# Autodesk Inventor assembly: SHPSNA5
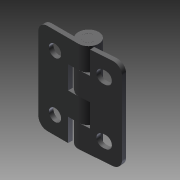
[picture p0: Inventor's stored thumbnail of the model, 180x180]
Saved by Autodesk Inventor 2015 SP1 (Build 190203100, 203)
## iProperties
Category: PARTsolutions
Company: MISUMI
Created: 2015-01-26
Part Number: SHPSNA5
Catalog Web Link: www.cadenas.de
Description: SHPSNA-Hinges with Slotted Holes
Vendor: MISUMI
Document SubType Name: Assembly
Designer: PARTuser1
Manufacturer: MISUMI
PSOL_IDENT_0: {\\10.0.0.236\data_v8\23d-libs\misumi\metric\44_handles_hinges\shpsna_asmtab.prj},161 {VTYP=3D},{STY
PSOL_IDENT_1: P=ASSTAB},{NB=SHPSNA5},{LINA=SHPSNA5},{NN=SHPSNA},{DATE=14.11.2014 09:15:25},{GEOMDATE=04.12.2008},{
PSOL_IDENT_2: VERSION=},{LINEID=10},{LINESUBID=-1},{WBVAR=}  {NB=SHPSNA5},{LINA=SHPSNA5},{KT=DUMMY},{PN=SHPSNA5},{
PSOL_IDENT_3: TYPE=SHPSNA},{MAT=304 Stainless Steel},{NO=5},{AL1=9},{AL2=88},{MASS=43},{L=41},{W=36},{K=8},{P=25},
PSOL_IDENT_4: {J=7.5},{S=21},{N=5.5},{Z=5.5x6.5},{Z1=5.5},{Z2=6.5},{T=2},{E=4.6},{R=4.6},{CR=4},{D=5},{PPATH=shpsn
PSOL_IDENT_5: a_asmtpl.prj}
SUPPLIER: MISUMI
ARTICLENO: SHPSNA5
BOMINFO: SHPSNA5
CREATOR: CADENAS GmbH
Title: SHPSNA5
Author: Cadenas PARTsolutions
Comments: Hinges with Slotted Holes
## Documents named in this file (4)
- C:\Users\Jack\ownCloud\Projects\CoreXY\InventorModel\Hardware\Hinges\HingeSHPSNA5\SHPSNA5.iam
- C:\Users\Jack\ownCloud\Projects\CoreXY\InventorModel\Hardware\Hinges\HingeSHPSNA5\SHPSNA5_1.ipt
- C:\Users\Jack\ownCloud\Projects\CoreXY\InventorModel\Hardware\Hinges\HingeSHPSNA5\SHPSNA5_2.ipt
- C:\Users\Jack\ownCloud\Projects\CoreXY\InventorModel\Hardware\Hinges\HingeSHPSNA5\SHPSNA5_3.ipt
## Components (3 placed, 3 different names)
1. SHPSNA5_1:1 — Mate:1, Flush:1
2. SHPSNA5_2:1 — Mate:1, Flush:1
3. SHPSNA5_3:1
## Relationships (2: Mate 1, Flush 1)
- Mate:1: SHPSNA5_1:1 ↔ SHPSNA5_2:1
- Flush:1: SHPSNA5_1:1 ↔ SHPSNA5_2:1
